(part 1 of 4)
# Autodesk Inventor assembly: 000 Ensamblaje hw_LM - BASIC
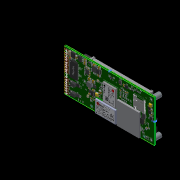
[picture p0: Inventor's stored thumbnail of the model, 180x180]
Saved by Autodesk Inventor 2018 (Build 220112000, 112)
## iProperties
Created: 2025-09-15
Part Number: 000 Ensamblaje hw_LM - BASIC
Document SubType Name: Assembly
Designer: mbs18
Mass: 915.711 g
Surface Area: 945.94 cm^2
Volume: 71.5532 cm^3
Density: 12.7976 g/cm^3
Author: mbs18
## Documents named in this file (64)
- C:\Users\mbs18.Embention\Git\LM\items\3d_LM\hw_LM\3d\000 Ensamblaje hw_LM - BASIC.iam
- C:\Users\mbs18.Embention\Git\LM\items\3d_LM\hw_LM\3d\hw_LM - PCB.ipt
- C:\Users\mbs18.Embention\Git\LM\items\_accesories\Componentes PCB\Tarjetero\3d_Molex\3d\47219-2001.ipt
- C:\Users\mbs18.Embention\Git\LM\items\_accesories\Componentes PCB\Magnetometro\3d_PNI Corp\3d\RM3100\Sen-XY-f.ipt
- C:\Users\mbs18.Embention\Git\LM\items\_accesories\Componentes PCB\Magnetometro\3d_PNI Corp\3d\RM3100\Sen-Z-f.ipt
- C:\Users\mbs18.Embention\Git\LM\items\_accesories\Componentes PCB\Conectores\3d_Samtec\3d\CLP-104-02-F-D-BE-TR.ipt
- C:\Users\mbs18.Embention\Git\LM\items\_accesories\Componentes PCB\Magnetometro\3d_PNI Corp\3d\RM3100\MAGI2C.ipt
- C:\Users\mbs18.Embention\Git\LM\items\_accesories\Componentes PCB\Resistencias\3d_Genérico\R0805.ipt
- C:\Users\mbs18.Embention\Git\LM\items\_accesories\Componentes PCB\Resistencias\3d_Mouser Electronics\3d\ERJ-U02F1601X\RES-1.6K_1%_0402.iam
- C:\Users\mbs18.Embention\Git\LM\items\_accesories\Componentes PCB\Conversores\CC-CC\3d_MuRata\3d\3d_MGJ1D121505MPC-R7\UND_0201CR___ _________.ipt
- C:\Users\mbs18.Embention\Git\LM\items\_accesories\Componentes PCB\Led\3d_ROHM EXCELED\3d\SML-D12V8WT86C.ipt
- C:\Users\mbs18.Embention\Git\LM\items\_accesories\Componentes PCB\Ferrita\3d_Murata Electronics\3d\BLM21PG220SN1D.ipt
- C:\Users\mbs18.Embention\Git\LM\items\_accesories\Componentes PCB\Capacitadores\3d_Kemet\3d\C1206C152KGRACAUTO.ipt
- C:\Users\mbs18.Embention\Git\LM\items\_accesories\Componentes PCB\Diodos\3d_Littlefuse\3d\AQ24CANFD-02HTG.ipt
- C:\Users\mbs18.Embention\Git\LM\items\_accesories\Componentes PCB\Jetson Orin Nano\Nvidia\Jetson_Orin_Nano_DevKit_3D_STEP_Model\095-0180-000-TS1_ASM.iam
- C:\Users\mbs18.Embention\Git\LM\items\_accesories\Componentes PCB\Microcontroladores\S32E288ABCAAMJGT.ipt
- C:\Users\mbs18.Embention\Git\LM\items\_accesories\Componentes PCB\Transceptor\3d_Texas Instrument\3d\DP83867ERGZT\DP83867ERGZT.iam
- C:\Users\mbs18.Embention\Git\LM\items\_accesories\Componentes PCB\CAN\3d\3d_Texas_Instruments\TCAN1462VDRBRQ1\TCAN1462VDRBRQ1.iam
- C:\Users\mbs18.Embention\Git\LM\items\_accesories\Componentes PCB\Diodos\3d_Bourns\3d\SMA6J64CA\SMA6J64CA.ipt
- C:\Users\mbs18.Embention\Git\LM\items\_accesories\Componentes PCB\Condensadores\3d_KEMET\3d\C1210C472KGRACAUTO\C1210C472KGRACAUTO.ipt
- C:\Users\mbs18.Embention\Git\LM\items\_accesories\Componentes PCB\Condensadores\3d_KEMET\3d\C0603C103K1RECAUTO\C0603C103K1RECAUTO.iam
- C:\Users\mbs18.Embention\Git\LM\items\_accesories\Componentes PCB\DC-DC\3d_Texas Instruments\3d\LM5146QRGYRQ1\LM5146QRGYRQ1.iam
- C:\Users\mbs18.Embention\Git\LM\items\_accesories\Componentes PCB\Bobinas\3d_COILCRAFT\3d\1812CAN-113NRC\1812CAN-113NRC.iam
- C:\Users\mbs18.Embention\Git\LM\items\_accesories\Componentes PCB\CAN\3d\Analog Devices\LTC2875MPDD#PBF.ipt
- C:\Users\mbs18.Embention\Git\LM\items\_accesories\Componentes PCB\Transceptor\3d_Texas Instrument\3d\UQFN-16.ipt
- C:\Users\mbs18.Embention\Git\LM\items\_accesories\Componentes PCB\Oscilador\3d_ECS_International\ECS-400-8-33Q-ADS-TR.ipt
- C:\Users\mbs18.Embention\Git\LM\items\_accesories\Componentes PCB\DC-DC\3d_Texas Instruments\3d\TPS3897ADRYT.ipt
- C:\Users\mbs18.Embention\Git\LM\items\_accesories\Componentes PCB\ESD Protection\3d_Nexperia\3d\PESD2CANFD27V-UX\PESD2CANFD27V-UX.iam
- C:\Users\mbs18.Embention\Git\LM\items\_accesories\Componentes PCB\Diodos\3d_Diodes Incorporated\3d\DMN2710UTQ-7\DMN2710UTQ-7.ipt
- C:\Users\mbs18.Embention\Git\LM\items\_accesories\Componentes PCB\Multiplexor\3d_TI\3d\SN74LVC1G08QDCKRQ1.ipt
- C:\Users\mbs18.Embention\Git\LM\items\_accesories\Componentes PCB\Bobinas\3d_COILCRAFT\3d\XAL7030-472MEC\XAL7030-472MEC.iam
- C:\Users\mbs18.Embention\Git\LM\items\_accesories\Componentes PCB\Inductor\3d_TDK\3d\XAL4020-601MEC\XAL4020-601MEC.ipt
- C:\Users\mbs18.Embention\Git\LM\items\_accesories\Componentes PCB\Diodos\3d_Texas Instrument\3d\TPD4E05U06QDQARQ1.ipt
- C:\Users\mbs18.Embention\Git\LM\items\_accesories\Componentes PCB\Diodos\3d_Littlefuse\3d\AQ05C-01FTG\AQ05C-01FTG.ipt
- C:\Users\mbs18.Embention\Git\LM\items\_accesories\Componentes PCB\GSM\3d_U-blox\3d\Sara\SARA.iam
- C:\Users\mbs18.Embention\Git\LM\items\_accesories\Componentes PCB\GPS - GNSS\3d_U-blox\3d\ZED F9P\u-blox ZED-F9P.ipt
- C:\Users\mbs18.Embention\Git\LM\items\_accesories\Ordenadores y Tablets\3d_NVIDIA\3d\Orin nano\Heatsink\ATS-NVP-3281-C2-R0.ipt
- C:\Users\mbs18.Embention\Git\LM\items\_accesories\Sensores\Sensor de presion\3d_Amphenol\3d\AUAV-L10D-M25125-RR-N.ipt
- C:\Users\mbs18.Embention\Git\LM\items\_accesories\Componentes PCB\Reguladores\3d_Analog\3d\LIB_LTC7103MPUHE#PBF\LTC7103MPUHE#PBF.ipt
- C:\Users\mbs18.Embention\Git\LM\items\_accesories\Componentes PCB\Active-low load\3d_Texas_Instruments\TPS22910AYZVR\Body.ipt
- C:\Users\mbs18.Embention\Git\LM\3d_LM - chapa.ipt
- C:\Users\mbs18.Embention\Git\LM\items\_accesories\Cables y conectores\3d_Hirose Electric Co Ltd\3d\UFL\U.FL-R-SMT-1.ipt
- C:\Users\mbs18.Embention\Git\LM\items\_accesories\Componentes PCB\Transformadores de señal\3d_Wurth Electroniks\3d\749020112B\749020112B.ipt
- C:\Users\mbs18.Embention\Git\LM\items\_accesories\Componentes PCB\Mosfet\3d_Vishay\3d\SQJ402EP-T1_GE3.ipt
- C:\Users\mbs18.Embention\Git\LM\items\_accesories\Componentes PCB\Condensadores\3d_KEMET\3d\T495B107M006ATE700\T495B107M006ATE700\T495B107M006ATE700.ipt
- C:\Users\mbs18.Embention\Git\LM\items\_accesories\Componentes PCB\Reguladores\3d_Texas Instruments\3d\TPS7A5301QRGRRQ1\TPS7A5301QRGRRQ1.iam
- C:\Users\mbs18.Embention\Git\LM\items\_accesories\Componentes PCB\SIM\3d_EMNIFY\3d\ESIM 638037665970.ipt
- C:\Users\mbs18.Embention\Git\LM\items\_accesories\Componentes PCB\Resistencias\3d_Kemet\3d\C0805X104K5RAC3316.ipt
- C:\Users\mbs18.Embention\Git\LM\items\_accesories\Componentes PCB\Reguladores\3d_Texas Instruments\3d\TPS57112CQRTERQ1\TPS57112CQRTERQ1.iam
- C:\Users\mbs18.Embention\Git\LM\items\_accesories\Componentes PCB\Oscilador\3d_ECS_International\ECS-2520MVQ-250-CN-TR\ECS-2520MVQ-250-CN-TR.ipt
- C:\Users\mbs18.Embention\Git\LM\items\_accesories\Cables y conectores\3d_Te Connectivity\3d\2309411-1\2309409-2-1.ipt
- C:\Users\mbs18.Embention\Git\LM\items\_accesories\Componentes PCB\Rectificadores\3d_Vishay\3d\AU3PM-M3_86A.ipt
- C:\Users\mbs18.Embention\Git\LM\items\_accesories\Componentes PCB\Inductor\3d_Vishay\IHLP2020CZER2R2MA1\IHLP2020CZER220M11.ipt
- C:\Users\mbs18.Embention\Git\LM\items\_accesories\Componentes PCB\Schottky Diodes\3d_STMicroelectronics\3d\STPST8H100SFY.ipt
- C:\Users\mbs18.Embention\Git\LM\items\_accesories\Componentes PCB\Reguladores\3d_Texas Instruments\3d\TPS74501PQWDRBRQ1\TPS74501PQWDRBRQ1.iam
- C:\Users\mbs18.Embention\Git\LM\items\_accesories\Componentes PCB\IMU\3d_Bosch\3d\BMI088.ipt
- C:\Users\mbs18.Embention\Git\LM\items\_accesories\Componentes PCB\Jetson Orin Nano\Nvidia\Jetson_Orin_NX_Orin_Nano_Module_3D_STEP_Model_20230310\P3767-pcba-envelop_20230310-modificada.ipt
- C:\Users\mbs18.Embention\Git\LM\items\_accesories\Separadores y torretas\Internal\Steel\3d_Wurth\3d\9774027151R (M2,5x2,7).ipt
- C:\Users\mbs18.Embention\Git\LM\items\_accesories\Separadores y torretas\Internal\Steel\3d_Wurth\3d\9774090360R (M3x9).ipt
- C:\Users\mbs18.Embention\Git\LM\items\_accesories\Componentes PCB\Mosfet\3d_Onsemi\SOT-363-6_2P2X1P35_ONS.ipt
- C:\Users\mbs18.Embention\Git\LM\items\_accesories\Componentes PCB\IMU\3d_TDK\IAM-20680HT.ipt
- C:\Users\mbs18.Embention\Git\LM\items\_accesories\Componentes PCB\IMU\3d_STM\ASM330LHBG1TR.ipt
- C:\Users\mbs18.Embention\Git\LM\items\_accesories\Componentes PCB\DC-DC\3d_Murata\MGJ1D151505MPC\UND_0201CR___ _________.ipt
- C:\Users\mbs18.Embention\Git\LM\items\_accesories\Ordenadores y Tablets\3d_NVIDIA\3d\Orin nano\Cooling Kit for NVIDIA Jetson Xavier NX - screws-harness.ipt
## Components (702 placed, 62 different names)
1. 2309409-2-1:1 — Mate:230, Mate:231, Mate:232, Angle:184
2. hw_LM - PCB:1 — Mate:1, Flush:1, Flush:2, Mate:29, Angle:6, Mate:33, Mate:35, Mate:60, Mate:72, Mate:84, Mate:94, Mate:95, Mate:107, Mate:108, Mate:109, Mate:110, Mate:112, Mate:113, Mate:114, Mate:115, Mate:116, Mate:117, Mate:118, Angle:53, Mate:123, Mate:124, Mate:131, Mate:132, Angle:59, Mate:134, Angle:62, Mate:135, Angle:64, Mate:136, Mate:139, Mate:153, Mate:154, Mate:155, Angle:91, Mate:187, Mate:188, Mate:194, Angle:142, Mate:199, Angle:149, Mate:200, Mate:203, Mate:210, Mate:213, Mate:216, Mate:219, Mate:220, Mate:222, Mate:224, Mate:225, Mate:226, Mate:227, Flush:634, Mate:229, Mate:230, Mate:231, Mate:232, Mate:237, Angle:169, Mate:238, Mate:239, Mate:240, Mate:241, Mate:242, Mate:243, Mate:245, Mate:246, Mate:247, Mate:248, Angle:176, Mate:249, Angle:177, Angle:178, Mate:250, Mate:251, Angle:179, Mate:252, Mate:253, Mate:254, Angle:180, Mate:256, Angle:181, Angle:182, Mate:257, Mate:258, Angle:183, Mate:259, Mate:267, Mate:268, Mate:269, Mate:270, Angle:185, Mate:271, Mate:272, Mate:273, Mate:274, Angle:189, Mate:275, Mate:276, Angle:193, Mate:277, Mate:278, Angle:194, Mate:279, Mate:280, Mate:281, Mate:282, Angle:195, Angle:198, Mate:285, Mate:286, Mate:287
3. 095-0180-000-TS1_ASM:1 [sub-assembly]
4. 47219-2001:1 — Mate:29, Angle:6
5. Sen-XY-f:1 — Mate:35, Flush:16
6. Sen-Z-f:1 — Mate:33, Angle:142
7. Sen-XY-f:2 — Flush:16
8. MAGI2C:1 — Mate:60
9. UND_0201CR___ _________:2
10. BLM21PG220SN1D:4 — Mate:247, Angle:189
11. C1206C152KGRACAUTO:3 — Flush:221, Flush:222, Flush:677
12. S32E288ABCAAMJGT:1 — Mate:94
13. DP83867ERGZT:1 [sub-assembly] — Mate:95
14. SML-D12V8WT86C:2 — Mate:107, Flush:202, Flush:611
15. SML-D12V8WT86C:3 — Mate:108
16. SML-D12V8WT86C:4 — Mate:109
17. SML-D12V8WT86C:5 — Mate:110
18. SML-D12V8WT86C:6 — Flush:202
19. SMA6J64CA:1 — Mate:116, Angle:63
20. SMA6J64CA:2 — Mate:117
21. C1210C472KGRACAUTO:1 — Mate:118
22. C0603C103K1RECAUTO:9 [sub-assembly] — Angle:53, Flush:222, Flush:223
23. C0603C103K1RECAUTO:10 [sub-assembly] — Flush:221
24. C0603C103K1RECAUTO:11 [sub-assembly] — Flush:223
25. 1812CAN-113NRC:1 [sub-assembly] — Mate:123, Flush:635
26. TCAN1462VDRBRQ1:5 [sub-assembly] — Mate:124, Flush:625
27. C1210C472KGRACAUTO:11 — Flush:228, Flush:230, Flush:232
28. C1210C472KGRACAUTO:12 — Flush:228, Flush:230, Flush:232, Flush:629
29. LTC2875MPDD#PBF:1 — Mate:131, Flush:331
30. UQFN-16:1 — Mate:132, Angle:59
31. LTC2875MPDD#PBF:2 — Flush:331
32. TPS3897ADRYT:1 — Mate:134
33. PESD2CANFD27V-UX:1 [sub-assembly] — Angle:62, Mate:135, Angle:63, Flush:650
34. DMN2710UTQ-7:1 — Angle:64, Mate:136
35. C0603C103K1RECAUTO:13 [sub-assembly] — Flush:662
36. C0603C103K1RECAUTO:14 [sub-assembly] — Flush:336, Angle:175
37. C0603C103K1RECAUTO:15 [sub-assembly] — Flush:336, Flush:653, Flush:660
38. DMN2710UTQ-7:7 — Flush:423, Flush:603
39. DMN2710UTQ-7:8 — Flush:423
40. C0603C103K1RECAUTO:18 [sub-assembly]
41. C0603C103K1RECAUTO:19 [sub-assembly]
42. C0603C103K1RECAUTO:20 [sub-assembly]
43. C0603C103K1RECAUTO:21 [sub-assembly]
44. C0603C103K1RECAUTO:22 [sub-assembly]
45. C0603C103K1RECAUTO:23 [sub-assembly]
46. XAL7030-472MEC:2 [sub-assembly]
47. C1206C152KGRACAUTO:8
48. R0805:5
49. XAL4020-601MEC:3 — Mate:188, Flush:627
50. TPD4E05U06QDQARQ1:1 — Mate:153, Flush:447
51. TPD4E05U06QDQARQ1:2 — Flush:448
52. TPD4E05U06QDQARQ1:3 — Flush:447, Flush:448, Flush:614
53. SARA:1 [sub-assembly] — Mate:194, Angle:200
54. SN74LVC1G08QDCKRQ1:2 — Angle:178
55. DMN2710UTQ-7:10 — Flush:603
56. LTC7103MPUHE#PBF:1 — Mate:187
57. SML-D12V8WT86C:7 — Flush:611
58. 749020112B:1 — Mate:199, Angle:149
59. 749020112B:2 — Mate:200
60. AQ05C-01FTG:2
61. AQ24CANFD-02HTG:8 — Mate:203, Angle:198, Angle:201
62. TPD4E05U06QDQARQ1:4 — Flush:614, Flush:615
63. TPD4E05U06QDQARQ1:5 — Flush:615
64. SQJ402EP-T1_GE3:1 — Mate:210, Mate:238
65. TPD4E05U06QDQARQ1:6 — Mate:213
66. T495B107M006ATE700:3 — Mate:216, Flush:652, Angle:195
67. TCAN1462VDRBRQ1:6 [sub-assembly] — Flush:625
68. XAL4020-601MEC:6 — Flush:627
69. SQJ402EP-T1_GE3:2 — Mate:219, Mate:220, Angle:176
70. C1210C472KGRACAUTO:19 — Mate:222
71. C1210C472KGRACAUTO:20 — Flush:629
72. C0805X104K5RAC3316:3 — Flush:631, Angle:197
73. C0805X104K5RAC3316:4 — Flush:631
74. TPS57112CQRTERQ1:1 [sub-assembly] — Mate:224
75. C0805X104K5RAC3316:5 — Flush:632
76. C0805X104K5RAC3316:6 — Flush:632, Flush:655
77. AQ05C-01FTG:3 — Mate:225
78. ECS-2520MVQ-250-CN-TR:1 — Mate:226
79. TCAN1462VDRBRQ1:7 [sub-assembly] — Mate:227
80. AUAV-L10D-M25125-RR-N:2 — Mate:229
81. AU3PM-M3_86A:1 — Mate:237, Angle:169
82. TPS7A5301QRGRRQ1:2 [sub-assembly] — Mate:239, Angle:304
83. U.FL-R-SMT-1:1 — Mate:241
84. U.FL-R-SMT-1:2 — Mate:240, Angle:197
85. u-blox ZED-F9P:1 — Mate:242, Angle:186
86. 1812CAN-113NRC:3 [sub-assembly] — Flush:635
87. IHLP2020CZER220M11:1 — Mate:243
88. R0805:11 — Mate:245
89. CLP-104-02-F-D-BE-TR:1 — Mate:246
90. LM5146QRGYRQ1:1 [sub-assembly] — Mate:248, Angle:175
91. STPST8H100SFY:1 — Mate:249, Angle:177
92. R0805:12 — Flush:638, Angle:191
93. R0805:13 — Flush:638, Angle:191
94. ESIM 638037665970:1 — Mate:250
95. ECS-400-8-33Q-ADS-TR:1 — Mate:251, Angle:179
96. TPS74501PQWDRBRQ1:1 [sub-assembly] — Mate:252, Flush:640
97. TPS74501PQWDRBRQ1:2 [sub-assembly] — Flush:640
98. C0603C103K1RECAUTO:24 [sub-assembly] — Mate:254, Angle:180, Flush:657, Flush:665, Flush:666
99. C0603C103K1RECAUTO:25 [sub-assembly] — Mate:253
100. C0603C103K1RECAUTO:26 [sub-assembly] — Flush:642, Flush:657, Flush:667
101. C0603C103K1RECAUTO:27 [sub-assembly] — Flush:641, Flush:642
102. C0603C103K1RECAUTO:28 [sub-assembly] — Flush:641
103. RES-1.6K_1%_0402:323 [sub-assembly] — Flush:1141
104. RES-1.6K_1%_0402:324 [sub-assembly]
105. RES-1.6K_1%_0402:325 [sub-assembly]
106. RES-1.6K_1%_0402:326 [sub-assembly]
107. SN74LVC1G08QDCKRQ1:3 — Mate:256, Angle:181
108. DMN2710UTQ-7:11 — Angle:182, Mate:257, Mate:258, Flush:647
109. DMN2710UTQ-7:12 — Flush:646, Flush:647, Angle:184, Flush:656
110. DMN2710UTQ-7:13 — Flush:646, Angle:183
111. Body:1 — Mate:259, Flush:648
112. Body:2 — Flush:648
113. PESD2CANFD27V-UX:4 [sub-assembly] — Flush:650
114. 9774027151R (M2,5x2,7):1 — Mate:262, Mate:263
115. 9774027151R (M2,5x2,7):2 — Mate:260, Mate:261
116. 9774090360R (M3x9):1 — Mate:267, Mate:268, Flush:651
117. 9774090360R (M3x9):2 — Flush:651, Mate:269
118. 9774090360R (M3x9):3 — Mate:270, Mate:272
119. T495B107M006ATE700:5 — Flush:652
120. SOT-363-6_2P2X1P35_ONS:1 — Angle:185, Mate:271, Angle:186
121. C1210C472KGRACAUTO:21 — Mate:273, Angle:188
122. C1210C472KGRACAUTO:22 — Mate:274, Angle:188
123. T495B107M006ATE700:6 — Mate:275
124. BMI088:1 — Mate:276, Angle:193
125. C0603C103K1RECAUTO:29 [sub-assembly] — Flush:653, Flush:659
126. C1206C152KGRACAUTO:9 — Mate:277
127. C0603C103K1RECAUTO:30 [sub-assembly] — Flush:654
128. C0603C103K1RECAUTO:31 [sub-assembly] — Flush:654, Flush:655
129. Body:4 — Mate:278
130. DMN2710UTQ-7:14 — Flush:656, Angle:194
131. AQ05C-01FTG:4 — Mate:279, Mate:280
132. C0603C103K1RECAUTO:33 [sub-assembly] — Flush:659
133. IAM-20680HT:1 — Mate:281, Flush:671
134. ASM330LHBG1TR:1 — Mate:282
135. C0603C103K1RECAUTO:34 [sub-assembly] — Flush:660, Flush:661, Flush:663
136. C0603C103K1RECAUTO:35 [sub-assembly] — Flush:661
137. C0603C103K1RECAUTO:36 [sub-assembly] — Flush:662, Flush:663
138. C0603C103K1RECAUTO:37 [sub-assembly] — Flush:664
139. C0603C103K1RECAUTO:38 [sub-assembly] — Flush:664, Flush:665
140. C0603C103K1RECAUTO:39 [sub-assembly] — Flush:666, Flush:668
141. C0603C103K1RECAUTO:40 [sub-assembly] — Flush:667, Flush:1101, Flush:1106, Flush:1129
142. C0603C103K1RECAUTO:41 [sub-assembly] — Flush:668
143. RES-1.6K_1%_0402:327 [sub-assembly] — Flush:669, Flush:670
144. RES-1.6K_1%_0402:328 [sub-assembly] — Flush:670
145. IAM-20680HT:2 — Flush:671
146. RES-1.6K_1%_0402:329 [sub-assembly] — Flush:674, Flush:676
147. RES-1.6K_1%_0402:330 [sub-assembly] — Flush:675
148. RES-1.6K_1%_0402:331 [sub-assembly] — Flush:674, Flush:675
149. C1206C152KGRACAUTO:10 — Flush:677
150. R0805:14 — Mate:285
151. C0603C103K1RECAUTO:42 [sub-assembly] — Mate:286, Flush:678
152. C0603C103K1RECAUTO:44 [sub-assembly] — Flush:678
153. UND_0201CR___ _________:3 — Mate:287, Flush:690, Flush:709
154. UND_0201CR___ _________:4 — Flush:681
155. UND_0201CR___ _________:5 — Flush:679, Flush:683
156. UND_0201CR___ _________:6 — Flush:682, Flush:683, Flush:737, Flush:798
157. UND_0201CR___ _________:7 — Flush:680, Flush:691
158. UND_0201CR___ _________:8 — Flush:679, Flush:680, Flush:681, Flush:692, Flush:706, Flush:772
159. UND_0201CR___ _________:9 — Flush:682, Flush:689, Flush:690
160. UND_0201CR___ _________:10 — Flush:691, Flush:708
161. UND_0201CR___ _________:11 — Flush:689, Flush:692
162. UND_0201CR___ _________:12
163. UND_0201CR___ _________:13
164. UND_0201CR___ _________:14
165. UND_0201CR___ _________:15 — Flush:707
166. UND_0201CR___ _________:16
167. UND_0201CR___ _________:17
168. UND_0201CR___ _________:18 — Flush:707
169. UND_0201CR___ _________:19 — Flush:709
170. UND_0201CR___ _________:20 — Flush:706
171. UND_0201CR___ _________:21
172. UND_0201CR___ _________:22
173. UND_0201CR___ _________:23
174. UND_0201CR___ _________:24
175. UND_0201CR___ _________:25 — Flush:708
176. UND_0201CR___ _________:26
177. UND_0201CR___ _________:27
178. UND_0201CR___ _________:28
179. UND_0201CR___ _________:29
180. UND_0201CR___ _________:30 — Flush:735
181. UND_0201CR___ _________:31
182. UND_0201CR___ _________:32 — Flush:736
183. UND_0201CR___ _________:33 — Flush:737
184. UND_0201CR___ _________:34
185. UND_0201CR___ _________:35 — Flush:734
186. UND_0201CR___ _________:36 — Flush:1130
187. UND_0201CR___ _________:37
188. UND_0201CR___ _________:38
189. UND_0201CR___ _________:39 — Flush:799
190. UND_0201CR___ _________:40 — Flush:735, Flush:772
191. UND_0201CR___ _________:41
192. UND_0201CR___ _________:42
193. UND_0201CR___ _________:43 — Flush:769
194. UND_0201CR___ _________:44 — Flush:768
195. UND_0201CR___ _________:45
196. UND_0201CR___ _________:46
197. UND_0201CR___ _________:47
198. UND_0201CR___ _________:48 — Flush:734
199. UND_0201CR___ _________:49 — Flush:736, Flush:770
200. UND_0201CR___ _________:50 — Flush:794
201. UND_0201CR___ _________:51 — Flush:768
202. UND_0201CR___ _________:52
203. UND_0201CR___ _________:53
204. UND_0201CR___ _________:54
205. UND_0201CR___ _________:55
206. UND_0201CR___ _________:56
207. UND_0201CR___ _________:57 — Flush:770, Flush:797
208. UND_0201CR___ _________:58
209. UND_0201CR___ _________:59
210. UND_0201CR___ _________:60 — Flush:771, Flush:793
211. UND_0201CR___ _________:61
212. UND_0201CR___ _________:62
213. UND_0201CR___ _________:63
214. UND_0201CR___ _________:64 — Flush:792
215. UND_0201CR___ _________:65 — Flush:795
216. UND_0201CR___ _________:66
217. UND_0201CR___ _________:67 — Flush:771, Flush:796, Flush:798
218. UND_0201CR___ _________:68
219. UND_0201CR___ _________:69 — Flush:773
220. UND_0201CR___ _________:70 — Flush:797
221. UND_0201CR___ _________:71
222. UND_0201CR___ _________:72
223. UND_0201CR___ _________:73
224. UND_0201CR___ _________:74
225. UND_0201CR___ _________:75
226. UND_0201CR___ _________:76 — Flush:769
227. UND_0201CR___ _________:77 — Flush:773
228. UND_0201CR___ _________:78
229. UND_0201CR___ _________:79
230. UND_0201CR___ _________:80
231. UND_0201CR___ _________:81 — Flush:819
232. UND_0201CR___ _________:82 — Flush:792
233. UND_0201CR___ _________:83 — Flush:799
234. UND_0201CR___ _________:84 — Flush:794, Flush:823, Flush:860, Flush:889, Flush:1035
235. UND_0201CR___ _________:85
236. UND_0201CR___ _________:86
237. UND_0201CR___ _________:87
238. UND_0201CR___ _________:88 — Flush:793
239. UND_0201CR___ _________:89
240. UND_0201CR___ _________:90 — Flush:795
241. UND_0201CR___ _________:91
242. UND_0201CR___ _________:92 — Flush:796, Flush:818
243. UND_0201CR___ _________:93
244. UND_0201CR___ _________:94
245. UND_0201CR___ _________:95
246. UND_0201CR___ _________:96
247. UND_0201CR___ _________:97
248. UND_0201CR___ _________:98
249. UND_0201CR___ _________:99
250. UND_0201CR___ _________:100
251. UND_0201CR___ _________:101 — Flush:819
252. UND_0201CR___ _________:102
253. UND_0201CR___ _________:103
254. UND_0201CR___ _________:104
255. UND_0201CR___ _________:105
256. UND_0201CR___ _________:106
257. UND_0201CR___ _________:107
258. UND_0201CR___ _________:108 — Flush:818
259. UND_0201CR___ _________:109
260. UND_0201CR___ _________:110
261. UND_0201CR___ _________:111
262. UND_0201CR___ _________:112 — Angle:201, Angle:202, Flush:822, Flush:831
263. UND_0201CR___ _________:113 — Angle:203, Flush:821, Flush:822, Flush:823, Flush:832
264. UND_0201CR___ _________:114 — Angle:202, Angle:203, Flush:821, Flush:830
265. UND_0201CR___ _________:115 — Flush:833
266. UND_0201CR___ _________:116 — Flush:832
267. UND_0201CR___ _________:117 — Flush:830
268. UND_0201CR___ _________:118 — Flush:831, Flush:833
269. UND_0201CR___ _________:119
270. UND_0201CR___ _________:120
271. UND_0201CR___ _________:121
272. UND_0201CR___ _________:122 — Flush:861
273. UND_0201CR___ _________:123
274. UND_0201CR___ _________:124
275. UND_0201CR___ _________:125 — Flush:862
276. UND_0201CR___ _________:126
277. UND_0201CR___ _________:127
278. UND_0201CR___ _________:128
279. UND_0201CR___ _________:129 — Flush:860
280. UND_0201CR___ _________:130
281. UND_0201CR___ _________:131 — Flush:890
282. UND_0201CR___ _________:132 — Flush:861
283. UND_0201CR___ _________:133 — Flush:862
284. UND_0201CR___ _________:134
285. UND_0201CR___ _________:135
286. UND_0201CR___ _________:136
287. UND_0201CR___ _________:137
288. UND_0201CR___ _________:138
289. UND_0201CR___ _________:139 — Flush:890
290. UND_0201CR___ _________:140
291. UND_0201CR___ _________:141
292. UND_0201CR___ _________:142
293. UND_0201CR___ _________:143
294. UND_0201CR___ _________:144 — Flush:891, Flush:918
295. UND_0201CR___ _________:145
296. UND_0201CR___ _________:146 — Flush:920
297. UND_0201CR___ _________:147
298. UND_0201CR___ _________:148 — Flush:891
299. UND_0201CR___ _________:149 — Flush:889
300. UND_0201CR___ _________:150
301. UND_0201CR___ _________:151
302. UND_0201CR___ _________:152
303. UND_0201CR___ _________:153
304. UND_0201CR___ _________:154
305. UND_0201CR___ _________:155
306. UND_0201CR___ _________:156
307. UND_0201CR___ _________:157
308. UND_0201CR___ _________:158
309. UND_0201CR___ _________:159 — Flush:918, Flush:919
310. UND_0201CR___ _________:160
311. UND_0201CR___ _________:161
312. UND_0201CR___ _________:162 — Flush:921
313. UND_0201CR___ _________:163
314. UND_0201CR___ _________:164
315. UND_0201CR___ _________:165 — Flush:1036, Flush:1136
316. UND_0201CR___ _________:166
317. UND_0201CR___ _________:167 — Flush:920, Flush:949, Flush:973
318. UND_0201CR___ _________:168 — Flush:919
319. UND_0201CR___ _________:169
320. UND_0201CR___ _________:170 — Flush:953
321. UND_0201CR___ _________:171 — Flush:921, Flush:952
322. UND_0201CR___ _________:172
323. UND_0201CR___ _________:173
324. UND_0201CR___ _________:174
325. UND_0201CR___ _________:175 — Flush:950
326. UND_0201CR___ _________:176 — Flush:948, Flush:949
327. UND_0201CR___ _________:177
328. UND_0201CR___ _________:178 — Flush:952, Flush:974, Flush:998
329. UND_0201CR___ _________:179
330. UND_0201CR___ _________:180 — Flush:951
331. UND_0201CR___ _________:181
332. UND_0201CR___ _________:182 — Flush:953, Flush:976
333. UND_0201CR___ _________:183
334. UND_0201CR___ _________:184
335. UND_0201CR___ _________:185 — Flush:948
336. UND_0201CR___ _________:186
337. UND_0201CR___ _________:187 — Flush:951
338. UND_0201CR___ _________:188
339. UND_0201CR___ _________:189
340. UND_0201CR___ _________:190
341. UND_0201CR___ _________:191 — Flush:950
342. UND_0201CR___ _________:192
343. UND_0201CR___ _________:193 — Flush:973, Flush:976
344. UND_0201CR___ _________:194 — Flush:974
345. UND_0201CR___ _________:195 — Flush:975
346. UND_0201CR___ _________:196
347. UND_0201CR___ _________:197
348. UND_0201CR___ _________:198 — Flush:997
349. UND_0201CR___ _________:199
350. UND_0201CR___ _________:200
351. UND_0201CR___ _________:201 — Flush:996
352. UND_0201CR___ _________:202 — Flush:975
353. UND_0201CR___ _________:203
354. UND_0201CR___ _________:204
355. UND_0201CR___ _________:205
356. UND_0201CR___ _________:206
357. UND_0201CR___ _________:207 — Flush:997
358. UND_0201CR___ _________:208 — Flush:1009
359. UND_0201CR___ _________:209
360. UND_0201CR___ _________:210
361. UND_0201CR___ _________:211
362. UND_0201CR___ _________:212
363. UND_0201CR___ _________:213 — Flush:996
364. UND_0201CR___ _________:214
365. UND_0201CR___ _________:215
366. UND_0201CR___ _________:216
367. UND_0201CR___ _________:217
368. UND_0201CR___ _________:218 — Flush:998
369. UND_0201CR___ _________:219
370. UND_0201CR___ _________:220 — Flush:1008
371. UND_0201CR___ _________:221 — Flush:1008, Flush:1031
372. UND_0201CR___ _________:222
373. UND_0201CR___ _________:223 — Flush:1009
374. UND_0201CR___ _________:224
375. UND_0201CR___ _________:225 — Flush:1032
376. UND_0201CR___ _________:226 — Flush:1029
377. UND_0201CR___ _________:227
378. UND_0201CR___ _________:228
379. UND_0201CR___ _________:229 — Flush:1029, Flush:1069
380. UND_0201CR___ _________:230 — Flush:1033
381. UND_0201CR___ _________:231 — Flush:1034
382. UND_0201CR___ _________:232 — Flush:1030
383. UND_0201CR___ _________:233 — Flush:1031
384. UND_0201CR___ _________:234
385. UND_0201CR___ _________:235
386. UND_0201CR___ _________:236 — Flush:1028, Flush:1036
387. UND_0201CR___ _________:237 — Flush:1033, Flush:1035
388. UND_0201CR___ _________:238 — Flush:1028
389. UND_0201CR___ _________:239
390. UND_0201CR___ _________:240 — Flush:1030, Flush:1034
391. UND_0201CR___ _________:241
392. UND_0201CR___ _________:242 — Flush:1032
393. UND_0201CR___ _________:243
394. UND_0201CR___ _________:244
395. UND_0201CR___ _________:249
396. UND_0201CR___ _________:250
397. UND_0201CR___ _________:251
398. UND_0201CR___ _________:252
399. UND_0201CR___ _________:253
400. UND_0201CR___ _________:257
401. UND_0201CR___ _________:261
402. UND_0201CR___ _________:262
403. UND_0201CR___ _________:266 — Flush:1069
404. UND_0201CR___ _________:267
405. UND_0201CR___ _________:268
406. RES-1.6K_1%_0402:332 [sub-assembly] — Flush:1070, Flush:1078
407. RES-1.6K_1%_0402:333 [sub-assembly] — Flush:1070, Flush:1073, Flush:1075
408. RES-1.6K_1%_0402:334 [sub-assembly] — Flush:1071
409. RES-1.6K_1%_0402:335 [sub-assembly] — Flush:1071, Flush:1072, Flush:1100
410. RES-1.6K_1%_0402:336 [sub-assembly] — Flush:1074
411. RES-1.6K_1%_0402:337 [sub-assembly] — Flush:1075, Flush:1078, Flush:1079
412. RES-1.6K_1%_0402:338 [sub-assembly] — Flush:1077, Flush:1079, Flush:1080
413. RES-1.6K_1%_0402:339 [sub-assembly] — Flush:1074, Flush:1077
414. RES-1.6K_1%_0402:340 [sub-assembly] — Flush:1080, Flush:1082
415. RES-1.6K_1%_0402:341 [sub-assembly] — Flush:1081, Flush:1083, Flush:1091
416. RES-1.6K_1%_0402:342 [sub-assembly] — Flush:1081, Flush:1083
417. RES-1.6K_1%_0402:343 [sub-assembly] — Flush:1082, Flush:1132
418. RES-1.6K_1%_0402:344 [sub-assembly] — Flush:1091
419. RES-1.6K_1%_0402:345 [sub-assembly] — Flush:1090, Flush:1093
420. RES-1.6K_1%_0402:346 [sub-assembly] — Flush:1090, Flush:1116, Flush:1128, Flush:1140
421. RES-1.6K_1%_0402:347 [sub-assembly] — Flush:1092, Flush:1112, Flush:1117
422. RES-1.6K_1%_0402:348 [sub-assembly] — Flush:1099, Flush:1100, Flush:1119
423. RES-1.6K_1%_0402:349 [sub-assembly]
424. RES-1.6K_1%_0402:350 [sub-assembly]
425. RES-1.6K_1%_0402:351 [sub-assembly]
426. RES-1.6K_1%_0402:352 [sub-assembly] — Flush:1099
427. RES-1.6K_1%_0402:353 [sub-assembly]
428. C0603C103K1RECAUTO:45 [sub-assembly] — Flush:1104
429. C0603C103K1RECAUTO:46 [sub-assembly] — Flush:1103, Flush:1104
430. C0603C103K1RECAUTO:47 [sub-assembly] — Flush:1102, Flush:1103
431. C0603C103K1RECAUTO:48 [sub-assembly] — Flush:1101, Flush:1102
432. C0603C103K1RECAUTO:49 [sub-assembly] — Flush:1106, Angle:306
433. C0603C103K1RECAUTO:50 [sub-assembly] — Flush:1108, Angle:305, Angle:306
434. C0603C103K1RECAUTO:51 [sub-assembly] — Flush:1108
435. C0603C103K1RECAUTO:52 [sub-assembly] — Angle:304, Angle:305
436. RES-1.6K_1%_0402:354 [sub-assembly] — Flush:1110, Flush:1111
437. RES-1.6K_1%_0402:355 [sub-assembly] — Flush:1109, Flush:1110
438. RES-1.6K_1%_0402:356 [sub-assembly] — Flush:1111
439. RES-1.6K_1%_0402:357 [sub-assembly] — Flush:1109, Flush:1112
440. RES-1.6K_1%_0402:358 [sub-assembly]
441. RES-1.6K_1%_0402:359 [sub-assembly] — Flush:1116
442. RES-1.6K_1%_0402:360 [sub-assembly] — Flush:1118, Flush:1119
443. RES-1.6K_1%_0402:361 [sub-assembly] — Flush:1117, Flush:1118
444. RES-1.6K_1%_0402:362 [sub-assembly] — Flush:1125, Flush:1128
445. RES-1.6K_1%_0402:363 [sub-assembly] — Flush:1126
446. RES-1.6K_1%_0402:364 [sub-assembly] — Flush:1124, Flush:1127
447. RES-1.6K_1%_0402:365 [sub-assembly] — Flush:1127
448. RES-1.6K_1%_0402:366 [sub-assembly] — Flush:1124, Flush:1126
449. RES-1.6K_1%_0402:367 [sub-assembly] — Flush:1125
450. C0603C103K1RECAUTO:53 [sub-assembly] — Flush:1129
451. UND_0201CR___ _________:269 — Flush:1130
452. UND_0201CR___ _________:270 — Flush:1135
453. UND_0201CR___ _________:271 — Flush:1135, Flush:1136
454. RES-1.6K_1%_0402:368 [sub-assembly] — Flush:1132, Flush:1133, Flush:1134
455. RES-1.6K_1%_0402:369 [sub-assembly] — Flush:1134
456. RES-1.6K_1%_0402:370 [sub-assembly] — Flush:1133
457. RES-1.6K_1%_0402:371 [sub-assembly]
458. RES-1.6K_1%_0402:372 [sub-assembly] — Flush:1140
459. RES-1.6K_1%_0402:373 [sub-assembly] — Flush:1139
460. RES-1.6K_1%_0402:374 [sub-assembly] — Flush:1139
461. RES-1.6K_1%_0402:375 [sub-assembly] — Flush:1142
462. Cooling Kit for NVIDIA Jetson Xavier NX - screws-harness:1 — Flush:1143, Mate:288, Mate:289
463. ATS-NVP-3281-C2-R0:1 — Mate:171
464. 3d_LM - chapa:1 — Mate:266, Mate:283, Mate:284
465. P3767-pcba-envelop_20230310-modificada:1 — Mate:154, Mate:155, Mate:171, Flush:634, Mate:260, Mate:261, Mate:262, Mate:263, Mate:266, Mate:283, Mate:284, Flush:1143, Mate:288, Mate:289
466. RES-1.6K_1%_0402:263 [sub-assembly] — Angle:95, Flush:517, Flush:535
467. RES-1.6K_1%_0402:1 [sub-assembly] — Mate:72
468. RES-1.6K_1%_0402:8 [sub-assembly] — Flush:59
469. RES-1.6K_1%_0402:9 [sub-assembly] — Flush:59
470. RES-1.6K_1%_0402:10 [sub-assembly]
471. RES-1.6K_1%_0402:13 [sub-assembly] — Flush:66
472. RES-1.6K_1%_0402:14 [sub-assembly] — Flush:64, Flush:65
473. RES-1.6K_1%_0402:15 [sub-assembly] — Flush:65, Flush:66
474. RES-1.6K_1%_0402:16 [sub-assembly] — Flush:64, Flush:73, Flush:118
475. RES-1.6K_1%_0402:18 [sub-assembly] — Flush:73
476. RES-1.6K_1%_0402:20 [sub-assembly]
477. RES-1.6K_1%_0402:21 [sub-assembly]
478. RES-1.6K_1%_0402:22 [sub-assembly] — Flush:85, Flush:86
479. RES-1.6K_1%_0402:25 [sub-assembly]
480. RES-1.6K_1%_0402:27 [sub-assembly] — Flush:85
481. RES-1.6K_1%_0402:28 [sub-assembly]
482. RES-1.6K_1%_0402:29 [sub-assembly] — Flush:86
483. RES-1.6K_1%_0402:31 [sub-assembly]
484. RES-1.6K_1%_0402:34 [sub-assembly]
485. RES-1.6K_1%_0402:35 [sub-assembly] — Flush:676
486. RES-1.6K_1%_0402:38 [sub-assembly]
487. RES-1.6K_1%_0402:40 [sub-assembly] — Flush:118
488. RES-1.6K_1%_0402:42 [sub-assembly]
489. RES-1.6K_1%_0402:44 [sub-assembly] — Flush:138
490. RES-1.6K_1%_0402:45 [sub-assembly]
491. RES-1.6K_1%_0402:48 [sub-assembly]
492. RES-1.6K_1%_0402:49 [sub-assembly]
493. RES-1.6K_1%_0402:50 [sub-assembly] — Flush:153
494. RES-1.6K_1%_0402:51 [sub-assembly] — Flush:153
495. RES-1.6K_1%_0402:53 [sub-assembly]
496. RES-1.6K_1%_0402:56 [sub-assembly] — Flush:138, Mate:84, Flush:146, Flush:151
497. RES-1.6K_1%_0402:58 [sub-assembly] — Flush:146
498. RES-1.6K_1%_0402:59 [sub-assembly] — Flush:151
499. RES-1.6K_1%_0402:60 [sub-assembly] — Flush:159
500. RES-1.6K_1%_0402:61 [sub-assembly] — Flush:160
501. RES-1.6K_1%_0402:62 [sub-assembly] — Flush:164, Flush:168
502. RES-1.6K_1%_0402:63 [sub-assembly] — Flush:159, Flush:160
503. RES-1.6K_1%_0402:64 [sub-assembly]
504. RES-1.6K_1%_0402:65 [sub-assembly] — Flush:164
505. RES-1.6K_1%_0402:66 [sub-assembly] — Flush:183
506. RES-1.6K_1%_0402:67 [sub-assembly] — Flush:182
507. RES-1.6K_1%_0402:69 [sub-assembly] — Flush:168
508. RES-1.6K_1%_0402:71 [sub-assembly]
509. RES-1.6K_1%_0402:72 [sub-assembly] — Flush:174
510. RES-1.6K_1%_0402:73 [sub-assembly]
511. RES-1.6K_1%_0402:75 [sub-assembly] — Flush:174
512. RES-1.6K_1%_0402:76 [sub-assembly] — Flush:183
513. RES-1.6K_1%_0402:77 [sub-assembly]
514. RES-1.6K_1%_0402:78 [sub-assembly] — Flush:186
515. RES-1.6K_1%_0402:79 [sub-assembly] — Flush:182
516. RES-1.6K_1%_0402:80 [sub-assembly] — Flush:186
517. RES-1.6K_1%_0402:81 [sub-assembly]
518. RES-1.6K_1%_0402:84 [sub-assembly] — Flush:192, Angle:199
519. RES-1.6K_1%_0402:85 [sub-assembly] — Flush:192, Flush:194
520. RES-1.6K_1%_0402:86 [sub-assembly] — Flush:194
521. RES-1.6K_1%_0402:88 [sub-assembly]
522. RES-1.6K_1%_0402:89 [sub-assembly] — Mate:115, Flush:204, Flush:205
523. RES-1.6K_1%_0402:90 [sub-assembly] — Mate:114, Flush:205, Flush:206
524. RES-1.6K_1%_0402:91 [sub-assembly] — Mate:113, Flush:206, Flush:207
525. RES-1.6K_1%_0402:92 [sub-assembly] — Mate:112, Flush:207
526. RES-1.6K_1%_0402:94 [sub-assembly] — Flush:204
527. RES-1.6K_1%_0402:97 [sub-assembly] — Mate:139, Flush:451, Flush:467, Flush:479, Flush:492, Flush:518
528. RES-1.6K_1%_0402:101 [sub-assembly]
529. RES-1.6K_1%_0402:104 [sub-assembly] — Flush:251
530. RES-1.6K_1%_0402:105 [sub-assembly] — Flush:252, Flush:261, Flush:278
531. RES-1.6K_1%_0402:107 [sub-assembly] — Flush:249, Flush:252
532. RES-1.6K_1%_0402:108 [sub-assembly]
533. RES-1.6K_1%_0402:109 [sub-assembly] — Flush:249, Flush:251
534. RES-1.6K_1%_0402:110 [sub-assembly]
535. RES-1.6K_1%_0402:113 [sub-assembly] — Flush:261, Flush:296, Flush:319
536. RES-1.6K_1%_0402:114 [sub-assembly]
537. RES-1.6K_1%_0402:115 [sub-assembly] — Flush:1142
538. RES-1.6K_1%_0402:117 [sub-assembly] — Flush:295
539. RES-1.6K_1%_0402:118 [sub-assembly]
540. RES-1.6K_1%_0402:120 [sub-assembly] — Flush:278
541. RES-1.6K_1%_0402:121 [sub-assembly]
542. RES-1.6K_1%_0402:123 [sub-assembly]
543. RES-1.6K_1%_0402:124 [sub-assembly]
544. RES-1.6K_1%_0402:128 [sub-assembly]
545. RES-1.6K_1%_0402:129 [sub-assembly]
546. RES-1.6K_1%_0402:130 [sub-assembly]
547. RES-1.6K_1%_0402:131 [sub-assembly]
548. RES-1.6K_1%_0402:132 [sub-assembly]
549. RES-1.6K_1%_0402:133 [sub-assembly]
550. RES-1.6K_1%_0402:134 [sub-assembly] — Flush:294
551. RES-1.6K_1%_0402:135 [sub-assembly]
552. RES-1.6K_1%_0402:136 [sub-assembly]
553. RES-1.6K_1%_0402:137 [sub-assembly] — Flush:296
554. RES-1.6K_1%_0402:138 [sub-assembly]
555. RES-1.6K_1%_0402:139 [sub-assembly] — Flush:294, Flush:295
556. RES-1.6K_1%_0402:140 [sub-assembly]
557. RES-1.6K_1%_0402:141 [sub-assembly]
558. RES-1.6K_1%_0402:142 [sub-assembly]
559. RES-1.6K_1%_0402:143 [sub-assembly] — Flush:327
560. RES-1.6K_1%_0402:144 [sub-assembly] — Flush:324
561. RES-1.6K_1%_0402:145 [sub-assembly] — Flush:317, Flush:328
562. RES-1.6K_1%_0402:146 [sub-assembly] — Flush:326, Flush:346
563. RES-1.6K_1%_0402:147 [sub-assembly] — Flush:318
564. RES-1.6K_1%_0402:148 [sub-assembly]
565. RES-1.6K_1%_0402:149 [sub-assembly]
566. RES-1.6K_1%_0402:150 [sub-assembly] — Flush:319
567. RES-1.6K_1%_0402:151 [sub-assembly]
568. RES-1.6K_1%_0402:155 [sub-assembly] — Flush:318
569. RES-1.6K_1%_0402:156 [sub-assembly]
570. RES-1.6K_1%_0402:157 [sub-assembly] — Flush:317
571. RES-1.6K_1%_0402:158 [sub-assembly]
572. RES-1.6K_1%_0402:159 [sub-assembly]
573. RES-1.6K_1%_0402:160 [sub-assembly] — Flush:326
574. RES-1.6K_1%_0402:161 [sub-assembly] — Flush:324, Flush:325, Flush:328
575. RES-1.6K_1%_0402:162 [sub-assembly] — Flush:325
576. RES-1.6K_1%_0402:164 [sub-assembly] — Flush:327
577. RES-1.6K_1%_0402:166 [sub-assembly]
578. RES-1.6K_1%_0402:168 [sub-assembly] — Flush:346
579. RES-1.6K_1%_0402:170 [sub-assembly] — Flush:382
580. RES-1.6K_1%_0402:178 [sub-assembly]
581. RES-1.6K_1%_0402:179 [sub-assembly]
582. RES-1.6K_1%_0402:180 [sub-assembly]
583. RES-1.6K_1%_0402:181 [sub-assembly]
584. RES-1.6K_1%_0402:182 [sub-assembly]
585. RES-1.6K_1%_0402:183 [sub-assembly] — Flush:382, Flush:383
586. RES-1.6K_1%_0402:184 [sub-assembly]
587. RES-1.6K_1%_0402:185 [sub-assembly] — Flush:384
588. RES-1.6K_1%_0402:186 [sub-assembly] — Angle:73, Angle:74
589. RES-1.6K_1%_0402:187 [sub-assembly] — Flush:386, Angle:74
590. RES-1.6K_1%_0402:188 [sub-assembly] — Flush:387, Angle:75
591. RES-1.6K_1%_0402:189 [sub-assembly] — Flush:388, Angle:71, Angle:72, Angle:75
592. RES-1.6K_1%_0402:190 [sub-assembly] — Angle:70, Angle:71
593. RES-1.6K_1%_0402:191 [sub-assembly] — Angle:69, Angle:70, Flush:398
594. RES-1.6K_1%_0402:192 [sub-assembly] — Angle:69
595. RES-1.6K_1%_0402:193 [sub-assembly] — Angle:72, Angle:73
596. RES-1.6K_1%_0402:194 [sub-assembly]
597. RES-1.6K_1%_0402:195 [sub-assembly] — Angle:199, Angle:200
598. RES-1.6K_1%_0402:196 [sub-assembly]
599. RES-1.6K_1%_0402:197 [sub-assembly] — Flush:386
600. RES-1.6K_1%_0402:198 [sub-assembly] — Flush:383
601. RES-1.6K_1%_0402:200 [sub-assembly] — Flush:384, Flush:388
602. RES-1.6K_1%_0402:201 [sub-assembly] — Flush:387
603. RES-1.6K_1%_0402:202 [sub-assembly] — Flush:398
604. RES-1.6K_1%_0402:203 [sub-assembly]
605. RES-1.6K_1%_0402:207 [sub-assembly]
606. RES-1.6K_1%_0402:208 [sub-assembly]
607. RES-1.6K_1%_0402:209 [sub-assembly]
608. RES-1.6K_1%_0402:210 [sub-assembly]
609. RES-1.6K_1%_0402:211 [sub-assembly]
610. RES-1.6K_1%_0402:212 [sub-assembly]
611. RES-1.6K_1%_0402:213 [sub-assembly]
612. RES-1.6K_1%_0402:214 [sub-assembly]
613. RES-1.6K_1%_0402:215 [sub-assembly] — Flush:417